# Autodesk Inventor assembly: Sarax_Quad
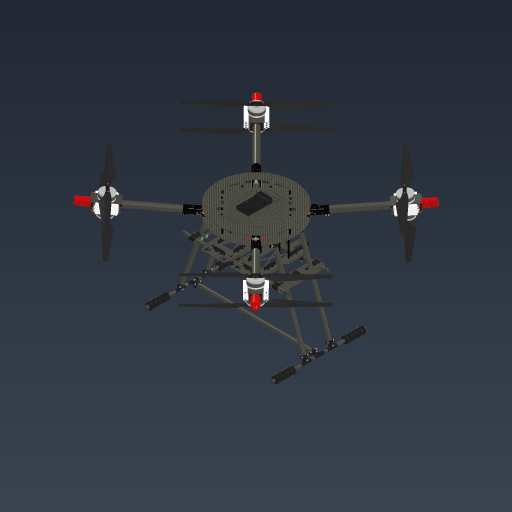
[picture p0: Inventor's stored thumbnail of the model, 512x512]
Saved by Autodesk Inventor 2024.1 (Build 281209000, 209)
## iProperties
RuleStatus: InUse
Created: 2023-12-05
Part Number: Sarax_Quad
Document SubType Name: Assembly
Designer: dzw04
Mass: 1945.83 g
Surface Area: 13465.8 cm^2
Volume: 1194.38 cm^3
Density: 1.62915 g/cm^3
Author: dzw04
## Documents named in this file (7)
- C:\Users\dzw04\Saxion\Mechatronica Lectoraat LMECH LED - Database ARG\Component_Database\SARAX\01. CAD\01. 3D_Drawing\Sarax_Quad.iam
- C:\Users\dzw04\Saxion\Mechatronica Lectoraat LMECH LED - Database ARG\Component_Database\SARAX\01. CAD\01. 3D_Drawing\02. Sub_Assemblies\Main_Body\Main_Body.iam
- C:\Users\dzw04\Saxion\Mechatronica Lectoraat LMECH LED - Database ARG\Component_Database\SARAX\01. CAD\01. 3D_Drawing\02. Sub_Assemblies\Core\Core.iam
- C:\Users\dzw04\Saxion\Mechatronica Lectoraat LMECH LED - Database ARG\Component_Database\SARAX\01. CAD\01. 3D_Drawing\02. Sub_Assemblies\Landing_Gear\Landing_Gear.iam
- C:\Users\dzw04\Saxion\Mechatronica Lectoraat LMECH LED - Database ARG\Component_Database\SARAX\01. CAD\01. 3D_Drawing\02. Sub_Assemblies\Arm\Arm.iam
- C:\Users\dzw04\Saxion\Mechatronica Lectoraat LMECH LED - Database ARG\Component_Database\SARAX\01. CAD\03. References\01. 3D_Files\PIXHAWK 5X-6X\PIXHAWK 5X-6X.ipt
- C:\Users\dzw04\Saxion\Mechatronica Lectoraat LMECH LED - Database ARG\Component_Database\SARAX\01. CAD\01. 3D_Drawing\Parameters.xlsx
## Components (8 placed, 5 different names)
1. Main_Body:1 [sub-assembly] — Mate:1, Mate:2, Mate:3, Mate:4, Mate:10, 3or6:1, 3or6:2, 4or8:1, 4or8:2, Mate:15, Mate:16, Angle:1
2. Core:1 [sub-assembly] — Mate:1, Mate:2, Mate:3, Flush:1, Mate:9, Mate:17, Flush:2, Flush:3
3. Landing_Gear:1 [sub-assembly] — Mate:4, Mate:15, Mate:16
4. PIXHAWK 5X-6X:1 — Mate:17, Flush:2, Flush:3
5. Arm:1 [sub-assembly] — Mate:10, 3or6:1, 3or6:2, 4or8:1, 4or8:2
6. Arm:2 [sub-assembly]
7. Arm:3 [sub-assembly]
8. Arm:4 [sub-assembly]
## Component patterns: (4 elements, first: Arm:1)
## Relationships (17: Mate 13, Flush 3, Angle 1)
- Mate:1: Main_Body:1 ↔ Core:1
- Mate:2: Main_Body:1 ↔ Core:1
- Mate:3: Main_Body:1 ↔ Core:1
- Mate:4: Main_Body:1 ↔ Landing_Gear:1
- Flush:1 (10 mm): Core:1
- Mate:9: Core:1
- Mate:10: Main_Body:1 ↔ Arm:1
- 3or6:1 [Mate]: Main_Body:1 ↔ Arm:1
- 3or6:2 [Mate]: Main_Body:1 ↔ Arm:1
- 4or8:1 [Mate]: Main_Body:1 ↔ Arm:1
- 4or8:2 [Mate]: Main_Body:1 ↔ Arm:1
- Mate:15: Main_Body:1 ↔ Landing_Gear:1
- Mate:16: Main_Body:1 ↔ Landing_Gear:1
- Angle:1 (0 deg): Main_Body:1
- Mate:17: Core:1 ↔ PIXHAWK 5X-6X:1
- Flush:2 (9.65 mm): Core:1 ↔ PIXHAWK 5X-6X:1
- Flush:3 (6.5 mm): Core:1 ↔ PIXHAWK 5X-6X:1
## Named parameters: BatteryWidth = 62 mm, BatteryLength = 200 mm, BatteryHeight = 76 mm, NumberOfArms = 4, RotorToRotor = 900 mm, MountToMotorCenter = 0 mm, ArmPosition = 5 deg, ThicknessBodyCenterPlate = 2 mm, ThicknessBodyOuterPlate = 2 mm, ThicknessLegLoadpipePlate = 2 mm, ThicknessBatteryTray = 2 mm, ThicknessBatteryTopTray = 1 mm, LoadpipeLength = 450 mm, NumberOfBatterys = 2, LandingGearHeight = 400 mm, LandingGearStabilityBar = 525 mm, LandingGearRod = 390 mm, StartAngleArm = 45 deg, ArmNr = 4, LGHeight = 400 mm, MotorToMotor = 900 mm, MotorToMountCenter = 71.5 mm, MotorMountCenter = 71.5 mm
